# Autodesk Inventor assembly: flip down main_MIR
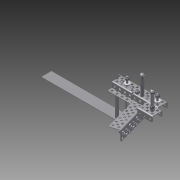
[picture p0: Inventor's stored thumbnail of the model, 180x180]
Saved by Autodesk Inventor 2014 SP1 (Build 180222100, 222)
## iProperties
Created: 2013-10-24
Part Number: flip down main_MIR
Document SubType Name: Assembly
Designer: RyanHughes
Author: RyanHughes
## Documents named in this file (20)
- C:\Users\Ryan\Desktop\sw\toss up 2ed A bot\intake\flip down main_MIR.iam
- C:\Users\Ryan\Desktop\sw\lib\Aperture VEX CAD Library\Bearing Blocks\Bearing Block.ipt
- C:\Users\Ryan\Desktop\sw\lib\Aperture VEX CAD Library\Hardware\8-32\8-32_.500.ipt
- C:\Users\Ryan\Desktop\sw\lib\Aperture VEX CAD Library\Metal\C Channel\2 x 9.ipt
- C:\Users\Ryan\Desktop\sw\lib\Aperture VEX CAD Library\Hardware\8-32\8-32 Nylock_MIR3.ipt
- C:\Users\Ryan\Desktop\sw\lib\Aperture VEX CAD Library\Hardware\8-32\8-32 Nylock.ipt
- C:\Users\Ryan\Desktop\sw\lib\Aperture VEX CAD Library\Spacers\thin\SPACER-0320-00625.ipt
- C:\Users\Ryan\Desktop\sw\lib\Aperture VEX CAD Library\Spacers\thin\SPACER-0320-0500.ipt
- C:\Users\Ryan\Desktop\sw\lib\Aperture VEX CAD Library\Hardware\8-32\8-32_.875.ipt
- C:\Users\Ryan\Desktop\sw\lib\Aperture VEX CAD Library\Hardware\8-32\8-32_.375.ipt
- C:\Users\Ryan\Desktop\sw\lib\Aperture VEX CAD Library\Hardware\8-32\8-32_.250.ipt
- C:\Users\Ryan\Desktop\sw\lib\Aperture VEX CAD Library\Standoffs\BEAM-1000.ipt
- C:\Users\Ryan\Desktop\sw\lib\Aperture VEX CAD Library\Metal\C Channel\2 x 3.ipt
- C:\Users\Ryan\Desktop\sw\lib\Aperture VEX CAD Library\Spacers\thin\SPACER-0320-0250.ipt
- C:\Users\Ryan\Desktop\sw\lib\Aperture VEX CAD Library\Hardware\8-32\8-32_1.000.ipt
- C:\Users\Ryan\Desktop\sw\lib\Aperture VEX CAD Library\Spacers\SPACER-0500-0125.ipt
- C:\Users\Ryan\Desktop\sw\lib\Aperture VEX CAD Library\Metal\L Bar\2 x 8.ipt
- C:\Users\Ryan\Desktop\sw\lib\Aperture VEX CAD Library\Standoffs\BEAM-2000.ipt
- C:\Users\Ryan\Desktop\sw\lib\Aperture VEX CAD Library\Metal\L Bar\2 x 5.ipt
- C:\Users\Ryan\Desktop\sw\toss up 2ed A bot\intake\buckies poly\big ball holder_MIR.ipt
## Components (53 placed, 19 different names)
1. Bearing Block:1 — Mate:10, Mate:11, Mate:2, Mate:9, Mate:5, Mate:4, Mate:25, Mate:24, Mate:72, Mate:71
2. Bearing Block:2 — Mate:13, Mate:12, Mate:1, Mate:8, Mate:7, Mate:6, Mate:19, Mate:20, Mate:68, Mate:66
3. 8-32_.500:1 — Mate:10, Mate:14, Mate:23
4. 8-32_.500:2 — Mate:13, Mate:16, Mate:18
5. 8-32_.500:3 — Mate:11, Mate:15, Mate:22
6. 8-32_.500:4 — Mate:12, Mate:17, Mate:21
7. 2 x 9:1 — Mate:17, Mate:16, Mate:15, Mate:14, Mate:2, Mate:1, Mate:9, Mate:8, Mate:7, Mate:6, Mate:5, Mate:4, Mate:30, Mate:29, Mate:28, Mate:36, Mate:52, Mate:51, Mate:50, Mate:54, Flush:2, Flush:1, Mate:55, Mate:65, Mate:70, Mate:93, Flush:4, Flush:5
8. 8-32 Nylock_MIR3:1 — Mate:19, Mate:18
9. 8-32 Nylock:1 — Mate:21, Mate:20
10. 8-32 Nylock:2 — Mate:25, Mate:23
11. 8-32 Nylock:3 — Mate:24, Mate:22
12. SPACER-0320-00625:1 — Mate:27, Mate:26, Mate:33
13. SPACER-0320-0500:1 — Mate:30, Mate:29, Mate:28, Mate:27, Mate:26, Mate:31, Mate:37, Mate:86
14. 2 x 8:1 — Mate:33, Mate:31, Mate:38, Mate:42, Mate:40, Mate:45, Mate:44, Mate:49, Mate:48, Mate:86, Mate:87, Mate:88, Mate:90, Mate:91, Mate:92
15. 8-32 Nylock:4 — Mate:36, Mate:39
16. 8-32_.875:1 — Mate:39, Mate:38, Mate:37
17. 8-32_.250:1 — Mate:52, Mate:51, Mate:50, Mate:53
18. BEAM-1000:1 — Mate:54, Mate:53, Mate:64, Mate:63
19. 2 x 3:1 — Flush:2, Flush:1, Mate:55, Mate:58, Mate:57, Mate:56, Mate:80
20. 8-32_.250:2 — Mate:58, Mate:57, Mate:56, Mate:78, Mate:79
21. SPACER-0320-0500:2 — Mate:64, Mate:63, Mate:61, Mate:59, Mate:60
22. SPACER-0320-0250:1 — Mate:61, Mate:59, Mate:62, Mate:88
23. SPACER-0320-00625:2 — Mate:62, Mate:60, Mate:89
24. 8-32_1.000:1 — Mate:68, Mate:67, Mate:74
25. SPACER-0500-0125:1 — Mate:67, Mate:66, Mate:65, Mate:73
26. 8-32_1.000:2 — Mate:72, Mate:69, Mate:76
27. SPACER-0500-0125:2 — Mate:71, Mate:70, Mate:69, Mate:75
28. 8-32 Nylock:7 — Mate:74, Mate:73
29. 8-32 Nylock:8 — Mate:76, Mate:75
30. 8-32 Nylock:9 — Mate:78, Mate:81, Mate:83, Mate:82
31. SPACER-0320-0250:2 — Mate:81, Mate:80, Mate:79, Mate:87
32. BEAM-1000:2 — Mate:83, Mate:82, Mate:85, Mate:84
33. 8-32 Nylock:10 — Mate:85, Mate:84, Mate:86
34. 8-32_.250:3 — Mate:87, Mate:86
35. 8-32_.250:4 — Mate:89, Mate:88
36. 8-32_.375:3 — Flush:3, Mate:91, Mate:92
37. 8-32 Nylock:11 — Mate:90
38. BEAM-2000:1 — Mate:94, Mate:95, Mate:96, Mate:105
39. 2 x 5:1 — Mate:93, Flush:4, Flush:5, Mate:94, Mate:95, Mate:96, Mate:97, Mate:98, Mate:99, Mate:100, Mate:101, Mate:102
40. BEAM-2000:2 — Mate:98, Mate:99, Mate:101, Mate:104, Mate:108
41. BEAM-2000:3 — Mate:97, Mate:100, Mate:102, Mate:103, Mate:106, Mate:107
42. 8-32_.375:6 — Mate:103, Mate:111
43. 8-32_.375:7 — Mate:104, Mate:109
44. 8-32_.375:8 — Mate:105, Mate:110
45. big ball holder_MIR:1 — Mate:106, Mate:107, Mate:108, Mate:109, Mate:110, Mate:111
46. 8-32 Nylock:6 — Mate:48, Mate:46
47. 8-32_.375:1 — Mate:42, Mate:40, Mate:46, Mate:87
48. 8-32 Nylock:5 — Mate:49, Mate:47
49. 8-32_.375:2 — Mate:45, Mate:44, Mate:47, Mate:88, Flush:3
50. 8-32 Nylock:12
51. 8-32_.375:4
52. 8-32 Nylock:13
53. 8-32_.375:5
## Component patterns: (2 elements, first: 8-32 Nylock:6 + 8-32_.375:1 + 8-32 Nylock:5 + 8-32_.375:2)
## Relationships (113: Mate 108, Flush 5)
- Mate:10: Bearing Block:1 ↔ 8-32_.500:1
- Mate:13: Bearing Block:2 ↔ 8-32_.500:2
- Mate:11: Bearing Block:1 ↔ 8-32_.500:3
- Mate:12: Bearing Block:2 ↔ 8-32_.500:4
- Mate:17: 8-32_.500:4 ↔ 2 x 9:1
- Mate:16: 8-32_.500:2 ↔ 2 x 9:1
- Mate:15: 8-32_.500:3 ↔ 2 x 9:1
- Mate:14: 8-32_.500:1 ↔ 2 x 9:1
- Mate:2: Bearing Block:1 ↔ 2 x 9:1
- Mate:1: Bearing Block:2 ↔ 2 x 9:1
- Mate:9 (2.3114 mm): Bearing Block:1 ↔ 2 x 9:1
- Mate:8 (2.3114 mm): Bearing Block:2 ↔ 2 x 9:1
- Mate:7 (2.3114 mm): Bearing Block:2 ↔ 2 x 9:1
- Mate:6 (2.3114 mm): Bearing Block:2 ↔ 2 x 9:1
- Mate:5 (2.3114 mm): Bearing Block:1 ↔ 2 x 9:1
- Mate:4 (2.3114 mm): Bearing Block:1 ↔ 2 x 9:1
- Mate:19: Bearing Block:2 ↔ 8-32 Nylock_MIR3:1
- Mate:18: 8-32_.500:2 ↔ 8-32 Nylock_MIR3:1
- Mate:21: 8-32_.500:4 ↔ 8-32 Nylock:1
- Mate:20: Bearing Block:2 ↔ 8-32 Nylock:1
- Mate:25: Bearing Block:1 ↔ 8-32 Nylock:2
- Mate:23: 8-32_.500:1 ↔ 8-32 Nylock:2
- Mate:24: Bearing Block:1 ↔ 8-32 Nylock:3
- Mate:22: 8-32_.500:3 ↔ 8-32 Nylock:3
- Mate:30: 2 x 9:1 ↔ SPACER-0320-0500:1
- Mate:29 (2.3114 mm): 2 x 9:1 ↔ SPACER-0320-0500:1
- Mate:28 (2.3114 mm): 2 x 9:1 ↔ SPACER-0320-0500:1
- Mate:27: SPACER-0320-00625:1 ↔ SPACER-0320-0500:1
- Mate:26: SPACER-0320-00625:1 ↔ SPACER-0320-0500:1
- Mate:33: SPACER-0320-00625:1 ↔ 2 x 8:1
- Mate:31 (2.3114 mm): SPACER-0320-0500:1 ↔ 2 x 8:1
- Mate:36: 2 x 9:1 ↔ 8-32 Nylock:4
- Mate:39: 8-32 Nylock:4 ↔ 8-32_.875:1
- Mate:38: 2 x 8:1 ↔ 8-32_.875:1
- Mate:37: SPACER-0320-0500:1 ↔ 8-32_.875:1
- Mate:42 (2.3114 mm): 2 x 8:1 ↔ 8-32_.375:1
- Mate:40 (1.5875 mm): 2 x 8:1 ↔ 8-32_.375:1
- Mate:45 (1.5875 mm): 2 x 8:1 ↔ 8-32_.375:2
- Mate:44 (2.3114 mm): 2 x 8:1 ↔ 8-32_.375:2
- Mate:49: 2 x 8:1 ↔ 8-32 Nylock:5
- Mate:47: 8-32 Nylock:5 ↔ 8-32_.375:2
- Mate:48: 2 x 8:1 ↔ 8-32 Nylock:6
- Mate:46: 8-32 Nylock:6 ↔ 8-32_.375:1
- Mate:52 (2.3114 mm): 2 x 9:1 ↔ 8-32_.250:1
- Mate:51: 2 x 9:1 ↔ 8-32_.250:1
- Mate:50 (2.3114 mm): 2 x 9:1 ↔ 8-32_.250:1
- Mate:54: 2 x 9:1 ↔ BEAM-1000:1
- Mate:53: 8-32_.250:1 ↔ BEAM-1000:1
- Flush:2: 2 x 9:1 ↔ 2 x 3:1
- Flush:1: 2 x 9:1 ↔ 2 x 3:1
- Mate:55: 2 x 9:1 ↔ 2 x 3:1
- Mate:58 (2.3114 mm): 2 x 3:1 ↔ 8-32_.250:2
- Mate:57 (2.3114 mm): 2 x 3:1 ↔ 8-32_.250:2
- Mate:56: 2 x 3:1 ↔ 8-32_.250:2
- Mate:64: BEAM-1000:1 ↔ SPACER-0320-0500:2
- Mate:63: BEAM-1000:1 ↔ SPACER-0320-0500:2
- Mate:61: SPACER-0320-0500:2 ↔ SPACER-0320-0250:1
- Mate:59: SPACER-0320-0500:2 ↔ SPACER-0320-0250:1
- Mate:62: SPACER-0320-0250:1 ↔ SPACER-0320-00625:2
- Mate:60: SPACER-0320-0500:2 ↔ SPACER-0320-00625:2
- Mate:68: Bearing Block:2 ↔ 8-32_1.000:1
- Mate:67: 8-32_1.000:1 ↔ SPACER-0500-0125:1
- Mate:66: Bearing Block:2 ↔ SPACER-0500-0125:1
- Mate:65: 2 x 9:1 ↔ SPACER-0500-0125:1
- Mate:72: Bearing Block:1 ↔ 8-32_1.000:2
- Mate:71: Bearing Block:1 ↔ SPACER-0500-0125:2
- Mate:70: 2 x 9:1 ↔ SPACER-0500-0125:2
- Mate:69: 8-32_1.000:2 ↔ SPACER-0500-0125:2
- Mate:74: 8-32_1.000:1 ↔ 8-32 Nylock:7
- Mate:73 (7.9375 mm): SPACER-0500-0125:1 ↔ 8-32 Nylock:7
- Mate:76: 8-32_1.000:2 ↔ 8-32 Nylock:8
- Mate:75 (7.9375 mm): SPACER-0500-0125:2 ↔ 8-32 Nylock:8
- Mate:78: 8-32_.250:2 ↔ 8-32 Nylock:9
- Mate:81: 8-32 Nylock:9 ↔ SPACER-0320-0250:2
- Mate:80: 2 x 3:1 ↔ SPACER-0320-0250:2
- Mate:79: 8-32_.250:2 ↔ SPACER-0320-0250:2
- Mate:83: 8-32 Nylock:9 ↔ BEAM-1000:2
- Mate:82: 8-32 Nylock:9 ↔ BEAM-1000:2
- Mate:85: BEAM-1000:2 ↔ 8-32 Nylock:10
- Mate:84: BEAM-1000:2 ↔ 8-32 Nylock:10
- Mate:87: SPACER-0320-0250:2 ↔ 8-32_.250:3
- Mate:86 (1.5875 mm): 8-32 Nylock:10 ↔ 8-32_.250:3
- Mate:89 (1.5875 mm): SPACER-0320-00625:2 ↔ 8-32_.250:4
- Mate:88: SPACER-0320-0250:1 ↔ 8-32_.250:4
- Mate:86 (2.3114 mm): SPACER-0320-0500:1 ↔ 2 x 8:1
- Mate:87 (2.3114 mm): 2 x 8:1 ↔ 8-32_.375:1
- Mate:88 (2.3114 mm): 2 x 8:1 ↔ 8-32_.375:2
- [Mate]: 8-32_.375:3 ↔ 8-32 Nylock:11
- Flush:3: 8-32_.375:3 ↔ 8-32_.375:2
- Mate:90: 2 x 8:1 ↔ 8-32 Nylock:11
- Mate:91 (2.3114 mm): 2 x 8:1 ↔ 8-32_.375:3
- Mate:92 (2.3114 mm): 2 x 8:1 ↔ 8-32_.375:3
- Mate:93: 2 x 9:1 ↔ 2 x 5:1
- Flush:4: 2 x 9:1 ↔ 2 x 5:1
- Flush:5: 2 x 9:1 ↔ 2 x 5:1
- Mate:94 (2.3114 mm): BEAM-2000:1 ↔ 2 x 5:1
- Mate:95: BEAM-2000:1 ↔ 2 x 5:1
- Mate:96 (2.3114 mm): BEAM-2000:1 ↔ 2 x 5:1
- Mate:97: 2 x 5:1 ↔ BEAM-2000:3
- Mate:98: 2 x 5:1 ↔ BEAM-2000:2
- Mate:99 (2.3114 mm): 2 x 5:1 ↔ BEAM-2000:2
- Mate:100 (2.3114 mm): 2 x 5:1 ↔ BEAM-2000:3
- Mate:101 (2.3114 mm): 2 x 5:1 ↔ BEAM-2000:2
- Mate:102 (2.3114 mm): 2 x 5:1 ↔ BEAM-2000:3
- Mate:103: BEAM-2000:3 ↔ 8-32_.375:6
- Mate:104: BEAM-2000:2 ↔ 8-32_.375:7
- Mate:105: BEAM-2000:1 ↔ 8-32_.375:8
- Mate:106: BEAM-2000:3 ↔ big ball holder_MIR:1
- Mate:107: BEAM-2000:3 ↔ big ball holder_MIR:1
- Mate:108: BEAM-2000:2 ↔ big ball holder_MIR:1
- Mate:109: 8-32_.375:7 ↔ big ball holder_MIR:1
- Mate:110: 8-32_.375:8 ↔ big ball holder_MIR:1
- Mate:111: 8-32_.375:6 ↔ big ball holder_MIR:1
## Named parameters: q = 2.3114 mm, d90_d45 = 0 mm
